# Autodesk Inventor assembly: assembled prototype car model
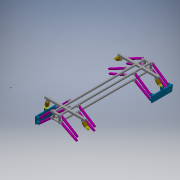
[picture p0: Inventor's stored thumbnail of the model, 180x180]
Saved by Autodesk Inventor 2016 (Build 200138000, 138)
## iProperties
Created: 2017-06-27
Part Number: assembled prototype car model
Document SubType Name: Assembly
Designer: andon
Author: andon
## Documents named in this file (8)
- E:\A human powered rover (Nasa)\Prototype\assembled prototype car model.iam
- E:\A human powered rover (Nasa)\Prototype\prototype body.ipt
- E:\A human powered rover (Nasa)\Prototype\wheel mount.ipt
- E:\A human powered rover (Nasa)\Prototype\body to wheel hub connectors (21 in).ipt
- E:\A human powered rover (Nasa)\Prototype\body to wheel hub connectors (19 in).ipt
- E:\A human powered rover (Nasa)\Prototype\shock absorber bottom.ipt
- E:\A human powered rover (Nasa)\Prototype\shock absorber top.ipt
- E:\A human powered rover (Nasa)\Prototype\screws.ipt
## Components (28 placed, 7 different names)
1. prototype body:1 — Mate:24, Mate:25, Mate:26, Flush:9, Mate:30, Mate:33, Mate:35, Mate:36, Mate:37, Mate:39, Mate:46, Mate:47, Mate:61, Mate:62, Mate:63, Mate:64, Mate:66, Mate:67, Mate:68, Flush:10, Mate:92, Mate:93, Mate:94, Mate:95, Mate:96, Mate:97, Mate:98, Mate:99, Mate:100, Mate:101, Mate:102, Mate:103, Mate:104, Mate:105, Mate:106
2. wheel mount:1 — Mate:28, Mate:31, Mate:34, Mate:40, Mate:41, Mate:42, Mate:43, Mate:44, Mate:45
3. body to wheel hub connectors (21 in):1 — Mate:24, Mate:35, Mate:36, Mate:40
4. body to wheel hub connectors (21 in):2 — Mate:25, Mate:26, Mate:28, Mate:42
5. body to wheel hub connectors (19 in):1 — Mate:30, Mate:31, Mate:33, Mate:43
6. body to wheel hub connectors (19 in):2 — Mate:34, Mate:37, Mate:39, Mate:41
7. shock absorber bottom:1 — Mate:44, Mate:45, Mate:48, Mate:49
8. shock absorber top:1 — Mate:46, Mate:47, Mate:48, Mate:49
9. body to wheel hub connectors (21 in):3 — Mate:63
10. body to wheel hub connectors (21 in):4 — Mate:61, Mate:66
11. body to wheel hub connectors (19 in):3 — Mate:62
12. body to wheel hub connectors (19 in):4 — Mate:64
13. shock absorber bottom:2 — Mate:59, Mate:60
14. shock absorber top:2 — Mate:59, Mate:60, Mate:67, Mate:68
15. body to wheel hub connectors (21 in):5 — Mate:95, Mate:103, Mate:105
16. body to wheel hub connectors (21 in):6 — Mate:100
17. body to wheel hub connectors (19 in):5 — Mate:101
18. body to wheel hub connectors (19 in):6 — Mate:102, Mate:104
19. shock absorber bottom:3 — Mate:78, Mate:79
20. shock absorber top:3 — Mate:78, Mate:79, Mate:94, Mate:106
21. wheel mount:4 — Mate:80, Mate:81, Mate:82, Mate:83, Mate:84, Mate:85, Mate:86, Mate:87, Mate:88, Mate:89
22. body to wheel hub connectors (21 in):7 — Mate:80, Mate:81, Mate:93, Mate:96
23. body to wheel hub connectors (21 in):8 — Mate:82, Mate:83, Mate:98
24. body to wheel hub connectors (19 in):7 — Mate:84, Mate:85, Mate:99
25. body to wheel hub connectors (19 in):8 — Mate:86, Mate:87, Mate:97
26. shock absorber bottom:4 — Mate:88, Mate:89, Mate:90, Mate:91
27. shock absorber top:4 — Mate:90, Mate:91, Mate:92
28. screws:1
## Relationships (62: Mate 60, Flush 2)
- Mate:24: prototype body:1 ↔ body to wheel hub connectors (21 in):1
- Mate:25: prototype body:1 ↔ body to wheel hub connectors (21 in):2
- Mate:26: prototype body:1 ↔ body to wheel hub connectors (21 in):2
- Mate:28: wheel mount:1 ↔ body to wheel hub connectors (21 in):2
- Flush:9: prototype body:1
- Mate:30: prototype body:1 ↔ body to wheel hub connectors (19 in):1
- Mate:31: wheel mount:1 ↔ body to wheel hub connectors (19 in):1
- Mate:33: prototype body:1 ↔ body to wheel hub connectors (19 in):1
- Mate:34: wheel mount:1 ↔ body to wheel hub connectors (19 in):2
- Mate:35: prototype body:1 ↔ body to wheel hub connectors (21 in):1
- Mate:36: prototype body:1 ↔ body to wheel hub connectors (21 in):1
- Mate:37: prototype body:1 ↔ body to wheel hub connectors (19 in):2
- Mate:39: prototype body:1 ↔ body to wheel hub connectors (19 in):2
- Mate:40: wheel mount:1 ↔ body to wheel hub connectors (21 in):1
- Mate:41: wheel mount:1 ↔ body to wheel hub connectors (19 in):2
- Mate:42: wheel mount:1 ↔ body to wheel hub connectors (21 in):2
- Mate:43: wheel mount:1 ↔ body to wheel hub connectors (19 in):1
- Mate:44: wheel mount:1 ↔ shock absorber bottom:1
- Mate:45: wheel mount:1 ↔ shock absorber bottom:1
- Mate:46: prototype body:1 ↔ shock absorber top:1
- Mate:47: prototype body:1 ↔ shock absorber top:1
- Mate:48: shock absorber bottom:1 ↔ shock absorber top:1
- Mate:49 (76.2 mm): shock absorber bottom:1 ↔ shock absorber top:1
- Mate:59 (76.2 mm): shock absorber bottom:2 ↔ shock absorber top:2
- Mate:60: shock absorber bottom:2 ↔ shock absorber top:2
- Mate:61: prototype body:1 ↔ body to wheel hub connectors (21 in):4
- Mate:62: prototype body:1 ↔ body to wheel hub connectors (19 in):3
- Mate:63: prototype body:1 ↔ body to wheel hub connectors (21 in):3
- Mate:64: prototype body:1 ↔ body to wheel hub connectors (19 in):4
- Mate:66: prototype body:1 ↔ body to wheel hub connectors (21 in):4
- Mate:67: prototype body:1 ↔ shock absorber top:2
- Mate:68: prototype body:1 ↔ shock absorber top:2
- Flush:10: prototype body:1
- Mate:78 (76.2 mm): shock absorber bottom:3 ↔ shock absorber top:3
- Mate:79: shock absorber bottom:3 ↔ shock absorber top:3
- Mate:80: wheel mount:4 ↔ body to wheel hub connectors (21 in):7
- Mate:81: wheel mount:4 ↔ body to wheel hub connectors (21 in):7
- Mate:82: wheel mount:4 ↔ body to wheel hub connectors (21 in):8
- Mate:83: wheel mount:4 ↔ body to wheel hub connectors (21 in):8
- Mate:84: wheel mount:4 ↔ body to wheel hub connectors (19 in):7
- Mate:85: wheel mount:4 ↔ body to wheel hub connectors (19 in):7
- Mate:86: wheel mount:4 ↔ body to wheel hub connectors (19 in):8
- Mate:87: wheel mount:4 ↔ body to wheel hub connectors (19 in):8
- Mate:88: wheel mount:4 ↔ shock absorber bottom:4
- Mate:89: wheel mount:4 ↔ shock absorber bottom:4
- Mate:90: shock absorber bottom:4 ↔ shock absorber top:4
- Mate:91 (76.2 mm): shock absorber bottom:4 ↔ shock absorber top:4
- Mate:92: prototype body:1 ↔ shock absorber top:4
- Mate:93: prototype body:1 ↔ body to wheel hub connectors (21 in):7
- Mate:94: prototype body:1 ↔ shock absorber top:3
- Mate:95: prototype body:1 ↔ body to wheel hub connectors (21 in):5
- Mate:96: prototype body:1 ↔ body to wheel hub connectors (21 in):7
- Mate:97: prototype body:1 ↔ body to wheel hub connectors (19 in):8
- Mate:98: prototype body:1 ↔ body to wheel hub connectors (21 in):8
- Mate:99: prototype body:1 ↔ body to wheel hub connectors (19 in):7
- Mate:100: prototype body:1 ↔ body to wheel hub connectors (21 in):6
- Mate:101: prototype body:1 ↔ body to wheel hub connectors (19 in):5
- Mate:102: prototype body:1 ↔ body to wheel hub connectors (19 in):6
- Mate:103: prototype body:1 ↔ body to wheel hub connectors (21 in):5
- Mate:104: prototype body:1 ↔ body to wheel hub connectors (19 in):6
- Mate:105: prototype body:1 ↔ body to wheel hub connectors (21 in):5
- Mate:106: prototype body:1 ↔ shock absorber top:3
